# Autodesk Inventor assembly: CORL_000_CoralAssembly
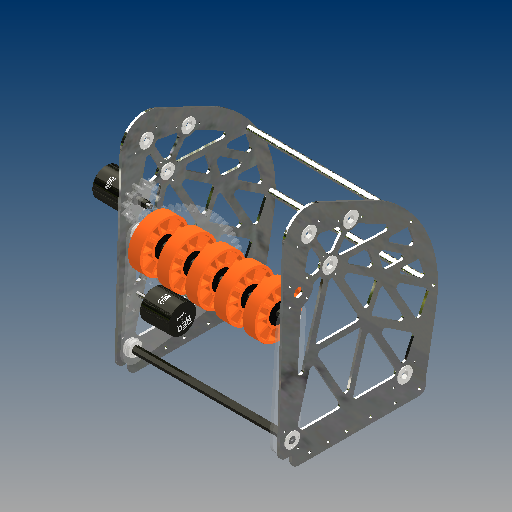
[picture p0: Inventor's stored thumbnail of the model, 512x512]
Saved by Autodesk Inventor 2024.3 (Build 283343000, 343)
## iProperties
Created: 2024-08-02
Part Number: CORL_000_CoralAssembly
Document SubType Name: Assembly
Designer: Bryan
Mass: 1860.11 g
Surface Area: 4686.68 cm^2
Volume: 1141.27 cm^3
Density: 1.62986 g/cm^3
Author: Bryan
## Documents named in this file (13)
- C:\Users\Kenji\Documents\GitHub\1622-2024-Summer-CAD-A-Thon\Coral\CORL_000_CoralAssembly.iam
- C:\Users\Kenji\Documents\GitHub\1622-2024-Summer-CAD-A-Thon\Coral\CORL_001_MainPlate.ipt
- C:\Users\Kenji\Documents\GitHub\1622-2024-Summer-CAD-A-Thon\COTS Library\Motion\Bearings\COTS_WCP-0783_1.125ODHexBearing.ipt
- C:\Users\Kenji\Documents\GitHub\1622-2024-Summer-CAD-A-Thon\Coral\CORL_002_FanPlate.ipt
- C:\Users\Kenji\Documents\GitHub\1622-2024-Summer-CAD-A-Thon\Coral\CORL_003_DropShaft.ipt
- C:\Users\Kenji\Documents\GitHub\1622-2024-Summer-CAD-A-Thon\Coral\CORL_004_PivotShaft.ipt
- C:\Users\Kenji\Documents\GitHub\1622-2024-Summer-CAD-A-Thon\Coral\CORL_005_PolyCarbSprocket.ipt
- C:\Users\Kenji\Documents\GitHub\1622-2024-Summer-CAD-A-Thon\COTS Library\Motion\Wheels\Compliant Wheels\4in compliant wheels\0.500in hex bore\COTS_am-3462_4indiameter_0.500inhexbore_durometer40A_CompliantWheel.ipt
- C:\Users\Kenji\Documents\GitHub\1622-2024-Summer-CAD-A-Thon\Coral\CORL_006_SmallPlate.ipt
- C:\Users\Kenji\Documents\GitHub\1622-2024-Summer-CAD-A-Thon\COTS Library\Motors\COTS_REV-21-1650-V1.1.ipt
- C:\Users\Kenji\Documents\GitHub\1622-2024-Summer-CAD-A-Thon\COTS Library\Adapters\COTS_REV-21-1879_8mmKeyTo0.5Hex.ipt
- C:\Users\Kenji\Documents\GitHub\1622-2024-Summer-CAD-A-Thon\Coral\CORL_008_MicroSpacer.ipt
- C:\Users\Kenji\Documents\GitHub\1622-2024-Summer-CAD-A-Thon\Coral\CORL_009_LongStandoff.ipt
## Components (33 placed, 12 different names)
1. CORL_001_MainPlate:1 — Mate:1, Mate:2, Mate:3, Mate:4, Mate:5, Mate:6, Mate:7, Mate:8, Mate:15, Mate:18, Mate:26, Mate:44, Mate:45, Mate:46, Mate:48
2. CORL_001_MainPlate:2 — Mate:1, Mate:2, Mate:3, Mate:9, Mate:10, Mate:11, Mate:12, Mate:13, Mate:29, Mate:47, Mate:65, Mate:66, Mate:67, Mate:68
3. COTS_WCP-0783_1.125ODHexBearing:1 — Mate:4, Flush:7
4. COTS_WCP-0783_1.125ODHexBearing:2 — Mate:5, Flush:6
5. COTS_WCP-0783_1.125ODHexBearing:3 — Mate:6, Flush:8
6. COTS_WCP-0783_1.125ODHexBearing:4 — Mate:7, Mate:26, Mate:30, Flush:2
7. COTS_WCP-0783_1.125ODHexBearing:5 — Mate:8, Mate:44, Flush:6, Flush:7, Flush:8
8. COTS_WCP-0783_1.125ODHexBearing:6 — Mate:9, Flush:9, Flush:10
9. COTS_WCP-0783_1.125ODHexBearing:7 — Mate:10, Mate:29, Flush:9
10. COTS_WCP-0783_1.125ODHexBearing:8 — Mate:11, Flush:12
11. COTS_WCP-0783_1.125ODHexBearing:9 — Mate:12, Flush:11, Flush:12
12. COTS_WCP-0783_1.125ODHexBearing:10 — Mate:13, Flush:10, Flush:11
13. CORL_002_FanPlate:2 — Mate:15, Mate:18, Mate:19, Mate:22, Mate:23, Mate:27, Mate:38, Flush:13, Mate:63, Flush:15, Mate:64
14. COTS_WCP-0783_1.125ODHexBearing:11 — Mate:19, Mate:27
15. COTS_WCP-0783_1.125ODHexBearing:12 — Mate:33, Flush:5, Mate:36, Mate:37
16. COTS_WCP-0783_1.125ODHexBearing:13 — Mate:32, Flush:4, Flush:5, Mate:35
17. COTS_WCP-0783_1.125ODHexBearing:14 — Mate:22, Mate:23, Mate:25
18. CORL_003_DropShaft:1 — Mate:25, Mate:32, Flush:4, Mate:34
19. CORL_004_PivotShaft:1 — Mate:30, Flush:2, Mate:33
20. CORL_006_SmallPlate:1 — Mate:35, Mate:36, Mate:37, Mate:47
21. COTS_REV-21-1650-V1.1:1 — Mate:45, Mate:46, Mate:48, Mate:56, Mate:57, Mate:61, Mate:62
22. CORL_008_MicroSpacer:1 — Mate:56, Mate:57
23. COTS_REV-21-1879_8mmKeyTo0.5Hex:2 — Mate:62, Flush:14
24. CORL_005_PolyCarbSprocket:3 — Mate:58, Mate:59, Mate:60, Flush:14
25. CORL_005_PolyCarbSprocket:4 — Mate:58, Mate:59, Mate:60, Mate:61, Flush:13
26. COTS_REV-21-1650-V1.1:2 — Mate:63, Flush:15, Mate:64
27. CORL_009_LongStandoff:1 — Mate:66, Mate:67
28. CORL_009_LongStandoff:2 — Mate:65, Mate:68
29. COTS_am-3462_4indiameter_0.500inhexbore_durometer40A_CompliantWheel:1 — Mate:34, Mate:38
30. COTS_am-3462_4indiameter_0.500inhexbore_durometer40A_CompliantWheel:2
31. COTS_am-3462_4indiameter_0.500inhexbore_durometer40A_CompliantWheel:3
32. COTS_am-3462_4indiameter_0.500inhexbore_durometer40A_CompliantWheel:4
33. COTS_am-3462_4indiameter_0.500inhexbore_durometer40A_CompliantWheel:5
## Component patterns: (5 elements, first: COTS_am-3462_4indiameter_0.500inhexbore_durometer40A_CompliantWheel:1)
## Relationships (61: Mate 48, Flush 13)
- Mate:1: CORL_001_MainPlate:1 ↔ CORL_001_MainPlate:2
- Mate:2: CORL_001_MainPlate:1 ↔ CORL_001_MainPlate:2
- Mate:3 (333.375 mm): CORL_001_MainPlate:1 ↔ CORL_001_MainPlate:2
- Mate:4: CORL_001_MainPlate:1 ↔ COTS_WCP-0783_1.125ODHexBearing:1
- Mate:5: CORL_001_MainPlate:1 ↔ COTS_WCP-0783_1.125ODHexBearing:2
- Mate:6: CORL_001_MainPlate:1 ↔ COTS_WCP-0783_1.125ODHexBearing:3
- Mate:7: CORL_001_MainPlate:1 ↔ COTS_WCP-0783_1.125ODHexBearing:4
- Mate:8: CORL_001_MainPlate:1 ↔ COTS_WCP-0783_1.125ODHexBearing:5
- Mate:9: CORL_001_MainPlate:2 ↔ COTS_WCP-0783_1.125ODHexBearing:6
- Mate:10: CORL_001_MainPlate:2 ↔ COTS_WCP-0783_1.125ODHexBearing:7
- Mate:11: CORL_001_MainPlate:2 ↔ COTS_WCP-0783_1.125ODHexBearing:8
- Mate:12: CORL_001_MainPlate:2 ↔ COTS_WCP-0783_1.125ODHexBearing:9
- Mate:13: CORL_001_MainPlate:2 ↔ COTS_WCP-0783_1.125ODHexBearing:10
- Mate:15: CORL_001_MainPlate:1 ↔ CORL_002_FanPlate:2
- Mate:18 (6.35 mm): CORL_001_MainPlate:1 ↔ CORL_002_FanPlate:2
- Mate:19: CORL_002_FanPlate:2 ↔ COTS_WCP-0783_1.125ODHexBearing:11
- Mate:22: CORL_002_FanPlate:2 ↔ COTS_WCP-0783_1.125ODHexBearing:14
- Mate:23: CORL_002_FanPlate:2 ↔ COTS_WCP-0783_1.125ODHexBearing:14
- Mate:25: COTS_WCP-0783_1.125ODHexBearing:14 ↔ CORL_003_DropShaft:1
- Mate:26: CORL_001_MainPlate:1 ↔ COTS_WCP-0783_1.125ODHexBearing:4
- Mate:27: CORL_002_FanPlate:2 ↔ COTS_WCP-0783_1.125ODHexBearing:11
- Mate:29: CORL_001_MainPlate:2 ↔ COTS_WCP-0783_1.125ODHexBearing:7
- Mate:30: COTS_WCP-0783_1.125ODHexBearing:4 ↔ CORL_004_PivotShaft:1
- Flush:2: COTS_WCP-0783_1.125ODHexBearing:4 ↔ CORL_004_PivotShaft:1
- Mate:32: COTS_WCP-0783_1.125ODHexBearing:13 ↔ CORL_003_DropShaft:1
- Flush:4: COTS_WCP-0783_1.125ODHexBearing:13 ↔ CORL_003_DropShaft:1
- Mate:33: COTS_WCP-0783_1.125ODHexBearing:12 ↔ CORL_004_PivotShaft:1
- Flush:5: COTS_WCP-0783_1.125ODHexBearing:12 ↔ COTS_WCP-0783_1.125ODHexBearing:13
- Mate:34: CORL_003_DropShaft:1 ↔ COTS_am-3462_4indiameter_0.500inhexbore_durometer40A_CompliantWheel:1
- Mate:35: COTS_WCP-0783_1.125ODHexBearing:13 ↔ CORL_006_SmallPlate:1
- Mate:36: COTS_WCP-0783_1.125ODHexBearing:12 ↔ CORL_006_SmallPlate:1
- Mate:37: COTS_WCP-0783_1.125ODHexBearing:12 ↔ CORL_006_SmallPlate:1
- Mate:38 (22.225 mm): CORL_002_FanPlate:2 ↔ COTS_am-3462_4indiameter_0.500inhexbore_durometer40A_CompliantWheel:1
- Mate:44: CORL_001_MainPlate:1 ↔ COTS_WCP-0783_1.125ODHexBearing:5
- Flush:6: COTS_WCP-0783_1.125ODHexBearing:2 ↔ COTS_WCP-0783_1.125ODHexBearing:5
- Flush:7: COTS_WCP-0783_1.125ODHexBearing:1 ↔ COTS_WCP-0783_1.125ODHexBearing:5
- Flush:8: COTS_WCP-0783_1.125ODHexBearing:3 ↔ COTS_WCP-0783_1.125ODHexBearing:5
- Flush:9: COTS_WCP-0783_1.125ODHexBearing:6 ↔ COTS_WCP-0783_1.125ODHexBearing:7
- Flush:10: COTS_WCP-0783_1.125ODHexBearing:6 ↔ COTS_WCP-0783_1.125ODHexBearing:10
- Flush:11: COTS_WCP-0783_1.125ODHexBearing:9 ↔ COTS_WCP-0783_1.125ODHexBearing:10
- Flush:12: COTS_WCP-0783_1.125ODHexBearing:8 ↔ COTS_WCP-0783_1.125ODHexBearing:9
- Mate:45: CORL_001_MainPlate:1 ↔ COTS_REV-21-1650-V1.1:1
- Mate:46: CORL_001_MainPlate:1 ↔ COTS_REV-21-1650-V1.1:1
- Mate:47 (6.35 mm): CORL_001_MainPlate:2 ↔ CORL_006_SmallPlate:1
- Mate:48: CORL_001_MainPlate:1 ↔ COTS_REV-21-1650-V1.1:1
- Mate:56: COTS_REV-21-1650-V1.1:1 ↔ CORL_008_MicroSpacer:1
- Mate:57: COTS_REV-21-1650-V1.1:1 ↔ CORL_008_MicroSpacer:1
- Mate:58: CORL_005_PolyCarbSprocket:3 ↔ CORL_005_PolyCarbSprocket:4
- Mate:59: CORL_005_PolyCarbSprocket:3 ↔ CORL_005_PolyCarbSprocket:4
- Mate:60: CORL_005_PolyCarbSprocket:3 ↔ CORL_005_PolyCarbSprocket:4
- Mate:61: COTS_REV-21-1650-V1.1:1 ↔ CORL_005_PolyCarbSprocket:4
- Flush:13 (-3.175 mm): CORL_002_FanPlate:2 ↔ CORL_005_PolyCarbSprocket:4
- Mate:62: COTS_REV-21-1650-V1.1:1 ↔ COTS_REV-21-1879_8mmKeyTo0.5Hex:2
- Flush:14: COTS_REV-21-1879_8mmKeyTo0.5Hex:2 ↔ CORL_005_PolyCarbSprocket:3
- Mate:63: CORL_002_FanPlate:2 ↔ COTS_REV-21-1650-V1.1:2
- Flush:15: CORL_002_FanPlate:2 ↔ COTS_REV-21-1650-V1.1:2
- Mate:64: CORL_002_FanPlate:2 ↔ COTS_REV-21-1650-V1.1:2
- Mate:65: CORL_001_MainPlate:2 ↔ CORL_009_LongStandoff:2
- Mate:66: CORL_001_MainPlate:2 ↔ CORL_009_LongStandoff:1
- Mate:67: CORL_001_MainPlate:2 ↔ CORL_009_LongStandoff:1
- Mate:68: CORL_001_MainPlate:2 ↔ CORL_009_LongStandoff:2
